# Autodesk Inventor assembly: PLC Casing Enclosure
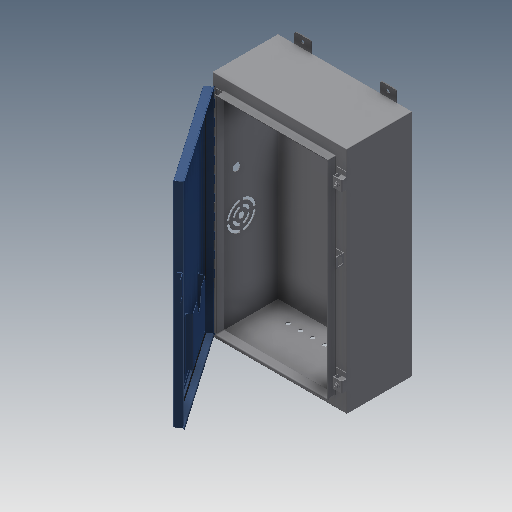
[picture p0: Inventor's stored thumbnail of the model, 512x512]
Saved by Autodesk Inventor 2019.1 (Build 231200000, 200)
## iProperties
Created: 2006-10-10
Part Number: PLC Casing Enclosure
Document SubType Name: Assembly
Designer: Administrator
Description: PLC Casing Enclosure
Stock Number: NA
Mass: 2642.23 g
Surface Area: 24498.8 cm^2
Volume: 2624.43 cm^3
Density: 1.00678 g/cm^3
Author: Administrator
Title: In House Assembly
Revision Number: A
## Documents named in this file (4)
- C:\Vault Workspace\Process Equipment\Workspace\Supplier Content\Electrical Design\Single Door Enclosure\PLC Casing Enclosure.iam
- C:\Vault Workspace\Process Equipment\Workspace\Supplier Content\Electrical Design\Single Door Enclosure\NEMA12 Enclosure.ipt
- C:\Vault Workspace\Process Equipment\Workspace\Supplier Content\Electrical Design\Single Door Enclosure\NEMA 12 Door.ipt
- C:\Vault Workspace\Process Equipment\Workspace\Supplier Content\Electrical Design\Single Door Enclosure\INSULATION-GASKET-2.ipt
## Components (3 placed, 3 different names)
1. NEMA12 Enclosure:1 — Insert:1, Mate:1, Mate:2
2. NEMA 12 Door:1 — Insert:1
3. INSULATION-GASKET-2:1 — Mate:1, Mate:2
## Relationships (3: Mate 2, Insert 1)
- Mate:1: NEMA12 Enclosure:1 ↔ INSULATION-GASKET-2:1
- Mate:2: NEMA12 Enclosure:1 ↔ INSULATION-GASKET-2:1
- Insert:1: NEMA12 Enclosure:1 ↔ NEMA 12 Door:1
